# Autodesk Inventor assembly: old_design_from_ebay
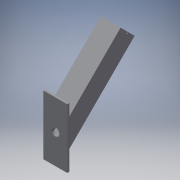
[picture p0: Inventor's stored thumbnail of the model, 180x180]
Saved by Autodesk Inventor 2018 (Build 220112000, 112)
## iProperties
Created: 2018-01-08
Part Number: old_design_from_ebay
Document SubType Name: Assembly
Designer: erwin
Author: erwin
## Documents named in this file (4)
- D:\GitHub\PrintableSpectroscope\design\old_design_from_ebay.iam
- D:\GitHub\PrintableSpectroscope\design\tube.ipt
- D:\GitHub\PrintableSpectroscope\design\base.ipt
- D:\GitHub\PrintableSpectroscope\design\top.ipt
## Components (3 placed, 3 different names)
1. tube:1 — Flush:1, Flush:2
2. base:1
3. top:1 — Flush:1, Flush:2
## Relationships (2: Flush 2)
- Flush:1: tube:1 ↔ top:1
- Flush:2: tube:1 ↔ top:1
